# Autodesk Inventor assembly: zadnji deo assebly
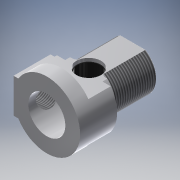
[picture p0: Inventor's stored thumbnail of the model, 180x180]
Saved by Autodesk Inventor 2019 (Build 230136000, 136)
## iProperties
Created: 2018-11-25
Part Number: zadnji deo assebly
Document SubType Name: Assembly
Designer: aleks
Author: aleks
## Documents named in this file (3)
- C:\Users\aleks\OneDrive\Desktop\novi klip\zadnji deo assebly.iam
- C:\Users\aleks\OneDrive\Desktop\novi klip\zadnji deo klipa.ipt
- C:\Users\aleks\OneDrive\Desktop\novi klip\ulozak.ipt
## Components (2 placed, 2 different names)
1. zadnji deo klipa:1 — Insert:1
2. ulozak:1 — Insert:1
## Relationships (1: Insert 1)
- Insert:1 (1 mm): zadnji deo klipa:1 ↔ ulozak:1
